# Autodesk Inventor assembly: Drone_stand
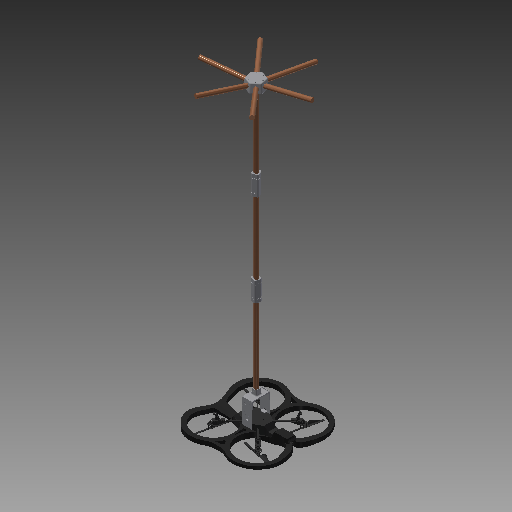
[picture p0: Inventor's stored thumbnail of the model, 512x512]
Saved by Autodesk Inventor 2019 (Build 230136000, 136)
## iProperties
Created: 2020-01-24
Part Number: Drone_stand
Document SubType Name: Assembly
Designer: Next
Author: Next
## Documents named in this file (8)
- C:\Users\Next\Desktop\My 3D Models\AR.Drone_2.0_stand\Drone_stand.iam
- C:\Users\Next\Desktop\My 3D Models\AR.Drone_2.0_stand\parts\Drone_holder_base.ipt
- C:\Users\Next\Desktop\My 3D Models\AR.Drone_2.0_stand\parts\Drone_holder_v1.1.ipt
- C:\Users\Next\Desktop\My 3D Models\AR.Drone_2.0_stand\parts\50cm_rod.ipt
- C:\Users\Next\Desktop\My 3D Models\AR.Drone_2.0_stand\AR.Drone_2.0_model\AR.Drone_2.0_Complete.iam
- C:\Users\Next\Desktop\My 3D Models\AR.Drone_2.0_stand\parts\Rod_base_v2.ipt
- C:\Users\Next\Desktop\My 3D Models\AR.Drone_2.0_stand\parts\25cm_rod.ipt
- C:\Users\Next\Desktop\My 3D Models\AR.Drone_2.0_stand\parts\Rod_Joint_v3.1.ipt
## Components (15 placed, 7 different names)
1. Drone_holder_v1.1:1 — Flush:2, Mate:1, Flush:3, Mate:7, Mate:8
2. Rod_Joint_v3.1:2 — Mate:9, Tangent:2, Mate:10, Tangent:3, Mate:13
3. Rod_Joint_v3.1:1 — Mate:11, Tangent:4, Mate:12, Tangent:5
4. Drone_holder_base:1 — Flush:2, Mate:1, Flush:3, Mate:2, Tangent:1
5. 50cm_rod:1 — Mate:2, Tangent:1, Mate:9, Tangent:2, Mate:13
6. 50cm_rod:2 — Mate:10, Tangent:3, Mate:11, Tangent:4
7. 50cm_rod:3 — Mate:12, Tangent:5, Mate:14, Tangent:6
8. AR.Drone_2.0_Complete:1 [sub-assembly] — Mate:7, Mate:8
9. Rod_base_v2:1 — Mate:14, Tangent:6, Mate:15, Tangent:7, Mate:16, Tangent:8, Mate:17, Tangent:9, Mate:18, Tangent:10, Mate:19, Tangent:11, Mate:20, Tangent:12
10. 25cm_rod:1 — Mate:16, Tangent:8
11. 25cm_rod:2 — Mate:18, Tangent:10
12. 25cm_rod:3 — Mate:17, Tangent:9
13. 25cm_rod:4 — Mate:15, Tangent:7
14. 25cm_rod:5 — Mate:19, Tangent:11
15. 25cm_rod:6 — Mate:20, Tangent:12
## Relationships (30: Mate 16, Tangent 12, Flush 2)
- Flush:2: Drone_holder_v1.1:1 ↔ Drone_holder_base:1
- Mate:1: Drone_holder_v1.1:1 ↔ Drone_holder_base:1
- Flush:3: Drone_holder_v1.1:1 ↔ Drone_holder_base:1
- Mate:2: Drone_holder_base:1 ↔ 50cm_rod:1
- Tangent:1: Drone_holder_base:1 ↔ 50cm_rod:1
- Mate:7: Drone_holder_v1.1:1 ↔ AR.Drone_2.0_Complete:1
- Mate:8: Drone_holder_v1.1:1 ↔ AR.Drone_2.0_Complete:1
- Mate:9: Rod_Joint_v3.1:2 ↔ 50cm_rod:1
- Tangent:2: Rod_Joint_v3.1:2 ↔ 50cm_rod:1
- Mate:10: Rod_Joint_v3.1:2 ↔ 50cm_rod:2
- Tangent:3: Rod_Joint_v3.1:2 ↔ 50cm_rod:2
- Mate:11: Rod_Joint_v3.1:1 ↔ 50cm_rod:2
- Tangent:4: Rod_Joint_v3.1:1 ↔ 50cm_rod:2
- Mate:12: Rod_Joint_v3.1:1 ↔ 50cm_rod:3
- Tangent:5: Rod_Joint_v3.1:1 ↔ 50cm_rod:3
- Mate:13: Rod_Joint_v3.1:2 ↔ 50cm_rod:1
- Mate:14: 50cm_rod:3 ↔ Rod_base_v2:1
- Tangent:6: 50cm_rod:3 ↔ Rod_base_v2:1
- Mate:15: Rod_base_v2:1 ↔ 25cm_rod:4
- Tangent:7: Rod_base_v2:1 ↔ 25cm_rod:4
- Mate:16: Rod_base_v2:1 ↔ 25cm_rod:1
- Tangent:8: Rod_base_v2:1 ↔ 25cm_rod:1
- Mate:17: Rod_base_v2:1 ↔ 25cm_rod:3
- Tangent:9: Rod_base_v2:1 ↔ 25cm_rod:3
- Mate:18: Rod_base_v2:1 ↔ 25cm_rod:2
- Tangent:10: Rod_base_v2:1 ↔ 25cm_rod:2
- Mate:19: Rod_base_v2:1 ↔ 25cm_rod:5
- Tangent:11: Rod_base_v2:1 ↔ 25cm_rod:5
- Mate:20: Rod_base_v2:1 ↔ 25cm_rod:6
- Tangent:12: Rod_base_v2:1 ↔ 25cm_rod:6
